# Autodesk Inventor assembly: Tor
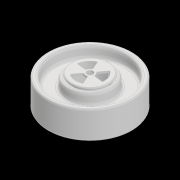
[picture p0: Inventor's stored thumbnail of the model, 180x180]
Saved by Autodesk Inventor 2020.4 (Build 244396010, 396A)
## iProperties
Created: 2022-09-18
Part Number: Tor
Document SubType Name: Assembly
Designer: Val
Author: Val
## Documents named in this file (3)
- C:\Users\Val\Desktop\tau\quote\Tor.iam
- C:\Users\Val\Desktop\tau\quote\TCore.ipt
- C:\Users\Val\Desktop\tau\quote\TCap.ipt
## Components (2 placed, 2 different names)
1. TCore:1 — Mate:1
2. TCap:1 — Mate:1
## Relationships (1: Mate 1)
- Mate:1: TCore:1 ↔ TCap:1
